# Autodesk Inventor assembly: Assembly_Cube_Z_Focus_MGN_NEMA_v3
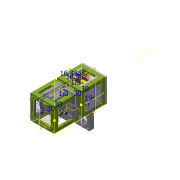
[picture p0: Inventor's stored thumbnail of the model, 180x180]
Saved by Autodesk Inventor 2022 (Build 260153000, 153)
## iProperties
Created: 2021-04-25
Part Number: Assembly_Cube_Z_Focus_MGN_NEMA_v3
Document SubType Name: Assembly
Designer: diederichbenedict
Author: diederichbenedict
## Documents named in this file (18)
- C:\Users\diederichbenedict\Dropbox\Dokumente\Promotion\PROJECTS\UC2\02_CAD\INVENTOR\uc2_v3\Assembly_Cube_Z_Focus_MGN_NEMA_v3.iam
- C:\Users\diederichbenedict\Dropbox\Dokumente\Promotion\PROJECTS\UC2\02_CAD\INVENTOR\uc2_v3\Assembly_Cube_empty_IM_v3.iam
- C:\Users\diederichbenedict\Dropbox\Dokumente\Promotion\PROJECTS\UC2\02_CAD\INVENTOR\uc2_v3\00_MGN12H, LINEAR GUIDE BLOCK.ipt
- C:\Users\diederichbenedict\Dropbox\Dokumente\Promotion\PROJECTS\UC2\02_CAD\INVENTOR\uc2_v3\00_NEMA11.ipt
- C:\Users\diederichbenedict\Dropbox\Dokumente\Promotion\PROJECTS\UC2\02_CAD\INVENTOR\uc2_v3\30_Cube_Z_Focus_MGN_NEMA_base_v3.ipt
- C:\Users\diederichbenedict\Dropbox\Dokumente\Promotion\PROJECTS\UC2\02_CAD\INVENTOR\uc2_v3\30_Cube_Z_Focus_MGN_NEMA_rail.ipt
- C:\Users\diederichbenedict\Dropbox\Dokumente\Promotion\PROJECTS\UC2\02_CAD\INVENTOR\uc2_v3\30_Cube_Z_Focus_Drylin_NEMA_slide_part1.ipt
- C:\Users\diederichbenedict\Dropbox\Dokumente\Promotion\PROJECTS\UC2\02_CAD\INVENTOR\uc2_v3\30_Cube_Z_Focus_MGN12_NEMA_slide_part2.ipt
- C:\Users\diederichbenedict\Dropbox\Dokumente\Promotion\PROJECTS\UC2\02_CAD\INVENTOR\uc2_v3\00_bearing_ball_2mm.ipt
- C:\Users\diederichbenedict\Dropbox\Dokumente\Promotion\PROJECTS\UC2\02_CAD\INVENTOR\uc2_v3\30_Cube_Z_Focus_MGN_NEMA_adapter_RMS.ipt
- C:\Users\diederichbenedict\Dropbox\Dokumente\Promotion\PROJECTS\UC2\02_CAD\INVENTOR\uc2_v3\Assembly_Motorcoupling_Nema_M3_Selfcentering.iam
- C:\Users\diederichbenedict\Dropbox\Dokumente\Promotion\PROJECTS\UC2\02_CAD\INVENTOR\uc2_v3\00_Stepper_Motor_28BYJ-48.ipt
- C:\Users\diederichbenedict\Dropbox\Dokumente\Promotion\PROJECTS\UC2\02_CAD\INVENTOR\uc2_v3\30_Cube_Z_Focus_MGN_NEMA_Motoradapter_NEMA11_v3.ipt
- C:\Users\diederichbenedict\Dropbox\Dokumente\Promotion\PROJECTS\UC2\02_CAD\INVENTOR\uc2_v3\30_Cube_Z_Focus_MGN_NEMA_Motoradapter_28BYJ_v3.ipt
- C:\Users\diederichbenedict\Dropbox\Dokumente\Promotion\PROJECTS\UC2\02_CAD\INVENTOR\uc2_v3\00_Motorcoupling_5mm_M3.ipt
- C:\Users\diederichbenedict\Dropbox\Dokumente\Promotion\PROJECTS\UC2\02_CAD\INVENTOR\uc2_v3\openSIMv3\BAK\30_Coupling_Screw_28BYJ_M3.ipt
- C:\Users\diederichbenedict\Dropbox\Dokumente\Promotion\PROJECTS\UC2\02_CAD\INVENTOR\uc2_v3\30_Cube_Z_Focus_MGN_NEMA_Motorsupport.ipt
- C:\Users\diederichbenedict\Dropbox\Dokumente\Promotion\PROJECTS\UC2\02_CAD\INVENTOR\uc2_v3\30_Cube_Z_Focus_MGN_NEMA_counterplate.ipt
## Components (21 placed, 17 different names)
1. Assembly_Motorcoupling_Nema_M3_Selfcentering:1 [sub-assembly]
2. 00_Stepper_Motor_28BYJ-48:1
3. 00_Motorcoupling_5mm_M3:2 — Einfügen:12
4. 30_Coupling_Screw_28BYJ_M3:1
5. 30_Cube_Z_Focus_MGN_NEMA_base_v3:1 — Mate:18, Mate:19, Mate:20, Insert:1, Insert:2, Insert:3, Insert:6
6. 00_Motorcoupling_5mm_M3:3 — Einfügen:8
7. 30_Cube_Z_Focus_MGN12_NEMA_slide_part2:1 — Fluchtend:2, Passend:23, Fluchtend:3, Einfügen:9, Einfügen:10
8. 30_Cube_Z_Focus_MGN_NEMA_adapter_RMS:1 — Einfügen:9
9. 00_MGN12H, LINEAR GUIDE BLOCK:1 — Passend:21, Passend:22, Fluchtend:1, Passend:23, Fluchtend:3
10. 30_Cube_Z_Focus_MGN_NEMA_rail:1 — Insert:6, Passend:22, Fluchtend:1
11. 30_Cube_Z_Focus_Drylin_NEMA_slide_part1:1 — Einfügen:10
12. 30_Cube_Z_Focus_MGN_NEMA_Motoradapter_NEMA11_v3:1 — Insert:3, Insert:4, Insert:5
13. 30_Cube_Z_Focus_MGN_NEMA_Motoradapter_28BYJ_v3:1 — Insert:1, Insert:2, Insert:4, Einfügen:12
14. 30_Cube_Z_Focus_MGN_NEMA_Motorsupport:1 — Passend:24, Passend:25
15. 00_bearing_ball_2mm:3
16. 00_bearing_ball_2mm:4
17. 00_bearing_ball_2mm:5
18. 00_NEMA11:1 — Insert:5, Einfügen:8
19. 30_Cube_Z_Focus_MGN_NEMA_counterplate:1 — Einfügen:11
20. Assembly_Cube_empty_IM_v3:4 [sub-assembly] — Mate:18, Mate:19, Mate:20, Passend:21, Fluchtend:2, Einfügen:11
21. Assembly_Cube_empty_IM_v3:6 [sub-assembly] — Passend:24, Passend:25
## Component patterns: (2 elements, first: Assembly_Cube_empty_IM_v3:4)
## Relationships (22: Insert 11, Mate 8, Flush 3)
- Mate:18: 30_Cube_Z_Focus_MGN_NEMA_base_v3:1 ↔ Assembly_Cube_empty_IM_v3:4
- Mate:19: 30_Cube_Z_Focus_MGN_NEMA_base_v3:1 ↔ Assembly_Cube_empty_IM_v3:4
- Mate:20: 30_Cube_Z_Focus_MGN_NEMA_base_v3:1 ↔ Assembly_Cube_empty_IM_v3:4
- Insert:1: 30_Cube_Z_Focus_MGN_NEMA_base_v3:1 ↔ 30_Cube_Z_Focus_MGN_NEMA_Motoradapter_28BYJ_v3:1
- Insert:2: 30_Cube_Z_Focus_MGN_NEMA_base_v3:1 ↔ 30_Cube_Z_Focus_MGN_NEMA_Motoradapter_28BYJ_v3:1
- Insert:3: 30_Cube_Z_Focus_MGN_NEMA_base_v3:1 ↔ 30_Cube_Z_Focus_MGN_NEMA_Motoradapter_NEMA11_v3:1
- Insert:4: 30_Cube_Z_Focus_MGN_NEMA_Motoradapter_NEMA11_v3:1 ↔ 30_Cube_Z_Focus_MGN_NEMA_Motoradapter_28BYJ_v3:1
- Insert:5: 30_Cube_Z_Focus_MGN_NEMA_Motoradapter_NEMA11_v3:1 ↔ 00_NEMA11:1
- Insert:6: 30_Cube_Z_Focus_MGN_NEMA_base_v3:1 ↔ 30_Cube_Z_Focus_MGN_NEMA_rail:1
- Einfügen:8 [Insert] (10 mm): 00_Motorcoupling_5mm_M3:3 ↔ 00_NEMA11:1
- Passend:21 [Mate]: 00_MGN12H, LINEAR GUIDE BLOCK:1 ↔ Assembly_Cube_empty_IM_v3:4
- Passend:22 [Mate]: 00_MGN12H, LINEAR GUIDE BLOCK:1 ↔ 30_Cube_Z_Focus_MGN_NEMA_rail:1
- Fluchtend:1 [Flush]: 00_MGN12H, LINEAR GUIDE BLOCK:1 ↔ 30_Cube_Z_Focus_MGN_NEMA_rail:1
- Fluchtend:2 [Flush]: 30_Cube_Z_Focus_MGN12_NEMA_slide_part2:1 ↔ Assembly_Cube_empty_IM_v3:4
- Passend:23 [Mate]: 30_Cube_Z_Focus_MGN12_NEMA_slide_part2:1 ↔ 00_MGN12H, LINEAR GUIDE BLOCK:1
- Fluchtend:3 [Flush]: 30_Cube_Z_Focus_MGN12_NEMA_slide_part2:1 ↔ 00_MGN12H, LINEAR GUIDE BLOCK:1
- Passend:24 [Mate]: 30_Cube_Z_Focus_MGN_NEMA_Motorsupport:1 ↔ Assembly_Cube_empty_IM_v3:6
- Passend:25 [Mate]: 30_Cube_Z_Focus_MGN_NEMA_Motorsupport:1 ↔ Assembly_Cube_empty_IM_v3:6
- Einfügen:9 [Insert]: 30_Cube_Z_Focus_MGN12_NEMA_slide_part2:1 ↔ 30_Cube_Z_Focus_MGN_NEMA_adapter_RMS:1
- Einfügen:10 [Insert]: 30_Cube_Z_Focus_MGN12_NEMA_slide_part2:1 ↔ 30_Cube_Z_Focus_Drylin_NEMA_slide_part1:1
- Einfügen:11 [Insert]: 30_Cube_Z_Focus_MGN_NEMA_counterplate:1 ↔ Assembly_Cube_empty_IM_v3:4
- Einfügen:12 [Insert]: 00_Motorcoupling_5mm_M3:2 ↔ 30_Cube_Z_Focus_MGN_NEMA_Motoradapter_28BYJ_v3:1
